# Autodesk Inventor assembly: mg996r 3mm foot_MIR
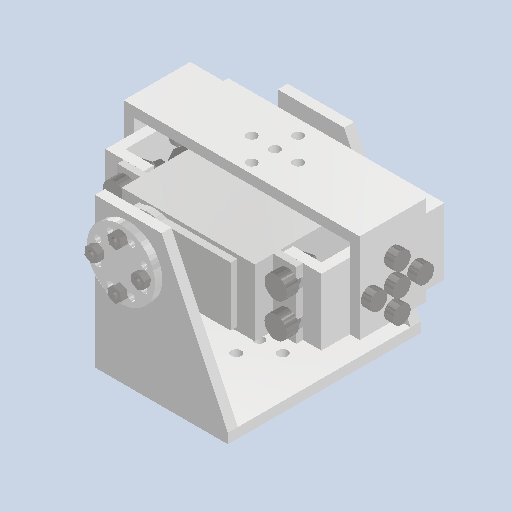
[picture p0: Inventor's stored thumbnail of the model, 512x512]
Saved by Autodesk Inventor 2023 (Build 270158000, 158)
## iProperties
Created: 2022-07-03
Part Number: mg996r 3mm foot_MIR
Document SubType Name: Assembly
Designer: isamu
Author: isamu
## iProperties of the stored document servo frame mg996r010.ipt
Created: 2022-07-03
Part Number: servo frame mg996r010
Material: Generic
Document SubType Name: Modeling
Designer: isamu
Density: 1 g/cm^3
Appearance: Default
Author: isamu
## iProperties of the stored document servo frame mg996 foot_MIR.iam
Created: 2022-07-03
Part Number: servo frame mg996 foot flipped
Description: FreeCAD Model
Document SubType Name: Assembly
Designer: isamu
Authority: Unknown
Sending System: FreeCAD
Preprocessor: Open CASCADE STEP processor 7.5
Title: Open CASCADE Shape Model
Author: Author
## Documents named in this file (8)
- D:\personal_projects\robot\inventor\mg996r 3mm foot_MIR.iam
- D:\personal_projects\robot\inventor\base mg996r 3mm with bottom.iam
- **D:\personal_projects\robot\inventor\mg996r 3mm foot_MIR.iam*LocalDocs*xAaaaqmaaAaaaaaaaAaaaarxuTb*servo frame mg996 foot_MIR.iam
- D:\personal_projects\robot\exports\frames\m2x8.ipt
- D:\personal_projects\robot\exports\frames\m2 nuts.ipt
- D:\personal_projects\robot\exports\frames\m4 nuts.ipt
- **D:\personal_projects\robot\inventor\mg996r 3mm foot_MIR.iam*LocalDocs*xAaaaapaaAaaaaaaaAaaaajunUh*servo frame mg996r010.ipt
- D:\personal_projects\robot\exports\frames\servo frame mg996 foot_MIR.step
## Components (11 placed, 5 different names)
1. base mg996r 3mm with bottom:1 [sub-assembly] — Mate:1, Mate:2, Mate:3, Insert:6, Insert:7, Insert:8, Insert:9
2. servo frame mg996 foot_MIR:1 [sub-assembly] — Mate:1, Mate:2, Mate:3, Insert:1, Insert:2, Insert:3, Insert:4, Insert:5
3. m2x8:1 — Insert:5
4. m2x8:2 — Insert:3
5. m2x8:3 — Insert:4
6. m2x8:4 — Insert:2
7. m2 nuts:1 — Insert:9
8. m2 nuts:2 — Insert:8
9. m2 nuts:3 — Insert:6
10. m2 nuts:4 — Insert:7
11. m4 nuts:1 — Insert:1
## Relationships (12: Insert 9, Mate 3)
- Mate:1: base mg996r 3mm with bottom:1 ↔ servo frame mg996 foot_MIR:1
- Mate:2: base mg996r 3mm with bottom:1 ↔ servo frame mg996 foot_MIR:1
- Mate:3: base mg996r 3mm with bottom:1 ↔ servo frame mg996 foot_MIR:1
- Insert:1: servo frame mg996 foot_MIR:1 ↔ m4 nuts:1
- Insert:2: servo frame mg996 foot_MIR:1 ↔ m2x8:4
- Insert:3: servo frame mg996 foot_MIR:1 ↔ m2x8:2
- Insert:4: servo frame mg996 foot_MIR:1 ↔ m2x8:3
- Insert:5: servo frame mg996 foot_MIR:1 ↔ m2x8:1
- Insert:6: base mg996r 3mm with bottom:1 ↔ m2 nuts:3
- Insert:7: base mg996r 3mm with bottom:1 ↔ m2 nuts:4
- Insert:8: base mg996r 3mm with bottom:1 ↔ m2 nuts:2
- Insert:9: base mg996r 3mm with bottom:1 ↔ m2 nuts:1
